# Autodesk Inventor assembly: module_top_icicles26_v2
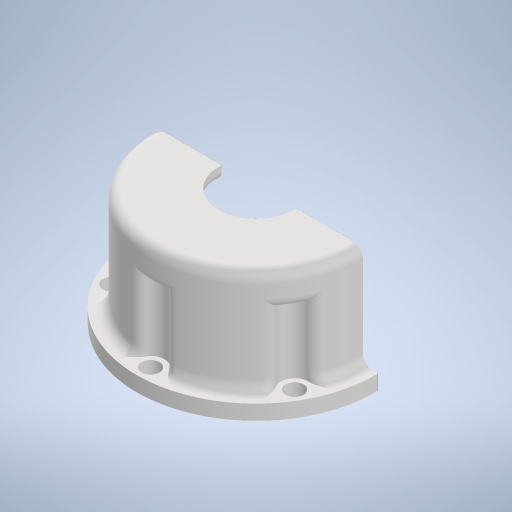
[picture p0: Inventor's stored thumbnail of the model, 512x512]
Saved by Autodesk Inventor 2023 (Build 270158000, 158)
## iProperties
Created: 2022-10-31
Part Number: module_top_icicles26_v2
Document SubType Name: Assembly
Designer: incep
Author: incep
## Documents named in this file (2)
- C:\Users\incep\OneDrive\Desktop\Laser Cutter Things\ModularUhOhChair\module_top_icicles26_v2.iam
- C:\Users\incep\OneDrive\Desktop\Laser Cutter Things\ModularUhOhChair\Module_top_Icicles26_v2.ipt
## Components (2 placed, 1 different names)
1. Module_top_Icicles26_v2:1 — Mate:1, Mate:2, Mate:3, Mate:6
2. Module_top_Icicles26_v2:2 — Mate:4, Mate:5, Mate:6
## Relationships (6: Mate 6)
- Mate:1: Module_top_Icicles26_v2:1
- Mate:2: Module_top_Icicles26_v2:1
- Mate:3: Module_top_Icicles26_v2:1
- Mate:4: Module_top_Icicles26_v2:2
- Mate:5: Module_top_Icicles26_v2:2
- Mate:6: Module_top_Icicles26_v2:1 ↔ Module_top_Icicles26_v2:2
